# Autodesk Inventor assembly: AdjusterAssembly
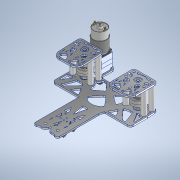
[picture p0: Inventor's stored thumbnail of the model, 180x180]
Saved by Autodesk Inventor 2020.2 (Build 242310000, 310)
## iProperties
Created: 2020-01-19
Part Number: AdjusterAssembly
Document SubType Name: Assembly
Designer: Paul Lefeuvre
Mass: 1604.28 g
Surface Area: 2645.53 cm^2
Volume: 583.424 cm^3
Density: 2.74977 g/cm^3
Author: Paul Lefeuvre
## Documents named in this file (10)
- C:\Users\Paul Lefeuvre\Documents\Inventor\7738-Adjuster\AdjusterAssembly.iam
- C:\Users\Paul Lefeuvre\Documents\Inventor\7738-Adjuster\CaseSheet.ipt
- C:\Users\Paul Lefeuvre\Documents\Inventor\7738-Adjuster\Colson_Performa_1_625_x_0_875_1_2_Hex_bore_217-4045.ipt
- C:\Users\Paul Lefeuvre\Documents\Inventor\7738-Adjuster\Axle1.ipt
- C:\Users\Paul Lefeuvre\Documents\Inventor\7738-Adjuster\F6800_Bearing.ipt
- C:\Users\Paul Lefeuvre\Documents\Inventor\7738-Adjuster\F6801_Bearing.ipt
- C:\Users\Paul Lefeuvre\Documents\Inventor\7738-Adjuster\MainHolder2.ipt
- C:\Users\Paul Lefeuvre\Documents\Inventor\7738-Adjuster\Spacer1.ipt
- C:\Users\Paul Lefeuvre\Documents\Inventor\7738-Adjuster\VersaPlanetary_v1_Single_Stage_10_1_with_775_Series.ipt
- C:\Users\Paul Lefeuvre\Documents\Inventor\7738-Adjuster\Mini V Gantry Kit.ipt
## Components (23 placed, 9 different names)
1. CaseSheet:1 — Insert:11, Mate:2, Mate:3, Mate:4
2. CaseSheet:2 — Insert:12, Insert:48, Insert:49, Insert:50, Insert:51
3. Colson_Performa_1_625_x_0_875_1_2_Hex_bore_217-4045:1 — Angle:1, Insert:2
4. Colson_Performa_1_625_x_0_875_1_2_Hex_bore_217-4045:2 — Angle:2, Insert:6
5. Axle1:1 — Angle:1, Angle:4, Insert:1, Insert:2, Insert:32, Insert:37
6. Axle1:2 — Angle:2, Angle:3, Insert:5, Insert:6, Insert:29, Insert:38
7. F6800_Bearing:1 — Insert:1, Insert:11
8. F6800_Bearing:2 — Insert:5, Insert:12
9. F6801_Bearing:1 — Insert:29
10. F6801_Bearing:2 — Insert:32
11. Colson_Performa_1_625_x_0_875_1_2_Hex_bore_217-4045:3 — Angle:3, Insert:38
12. Colson_Performa_1_625_x_0_875_1_2_Hex_bore_217-4045:4 — Angle:4, Insert:37
13. MainHolder2:1 — Flush:1, Mate:1, Insert:40, Insert:41, Insert:42, Insert:44, Insert:45, Insert:46, Mate:6, Mate:7, Angle:5, Insert:52, Insert:53, Insert:54, Insert:55, Insert:56, Insert:57
14. Spacer1:1 — Insert:40, Mate:3
15. Spacer1:2 — Insert:41, Mate:2
16. Spacer1:3 — Insert:42, Mate:4
17. Spacer1:4 — Insert:49
18. Spacer1:5 — Insert:44, Insert:50
19. Spacer1:6 — Insert:46, Insert:51
20. Spacer1:7 — Insert:52
21. Spacer1:8 — Insert:45, Insert:48
22. VersaPlanetary_v1_Single_Stage_10_1_with_775_Series:1 — Mate:6, Mate:7, Angle:5
23. Mini V Gantry Kit:1 — Insert:53, Insert:54, Insert:55, Insert:56, Insert:57
## Relationships (38: Insert 26, Mate 6, Angle 5, Flush 1)
- Angle:1 (0 deg): Colson_Performa_1_625_x_0_875_1_2_Hex_bore_217-4045:1 ↔ Axle1:1
- Angle:2 (0 deg): Colson_Performa_1_625_x_0_875_1_2_Hex_bore_217-4045:2 ↔ Axle1:2
- Angle:3 (0 deg): Axle1:2 ↔ Colson_Performa_1_625_x_0_875_1_2_Hex_bore_217-4045:3
- Angle:4 (0 deg): Axle1:1 ↔ Colson_Performa_1_625_x_0_875_1_2_Hex_bore_217-4045:4
- Insert:1 (0.6 mm): Axle1:1 ↔ F6800_Bearing:1
- Insert:2 (0.5 mm): Colson_Performa_1_625_x_0_875_1_2_Hex_bore_217-4045:1 ↔ Axle1:1
- Insert:5 (0.6 mm): Axle1:2 ↔ F6800_Bearing:2
- Insert:6 (0.5 mm): Colson_Performa_1_625_x_0_875_1_2_Hex_bore_217-4045:2 ↔ Axle1:2
- Insert:11 (0.6 mm): CaseSheet:1 ↔ F6800_Bearing:1
- Insert:12 (0.6 mm): CaseSheet:2 ↔ F6800_Bearing:2
- Insert:29 (0.6 mm): Axle1:2 ↔ F6801_Bearing:1
- Insert:32 (0.6 mm): Axle1:1 ↔ F6801_Bearing:2
- Insert:37 (0.5 mm): Axle1:1 ↔ Colson_Performa_1_625_x_0_875_1_2_Hex_bore_217-4045:4
- Insert:38 (0.5 mm): Axle1:2 ↔ Colson_Performa_1_625_x_0_875_1_2_Hex_bore_217-4045:3
- Flush:1: MainHolder2:1
- Mate:1: MainHolder2:1
- Insert:40 (0.75 mm): MainHolder2:1 ↔ Spacer1:1
- Insert:41 (0.75 mm): MainHolder2:1 ↔ Spacer1:2
- Insert:42 (0.75 mm): MainHolder2:1 ↔ Spacer1:3
- Insert:44 (0.75 mm): MainHolder2:1 ↔ Spacer1:5
- Mate:2 (0.75 mm): CaseSheet:1 ↔ Spacer1:2
- Mate:3 (0.75 mm): CaseSheet:1 ↔ Spacer1:1
- Mate:4 (0.75 mm): CaseSheet:1 ↔ Spacer1:3
- Insert:45 (0.75 mm): MainHolder2:1 ↔ Spacer1:8
- Insert:46 (0.75 mm): MainHolder2:1 ↔ Spacer1:6
- Insert:48 (0.75 mm): CaseSheet:2 ↔ Spacer1:8
- Insert:49 (0.75 mm): CaseSheet:2 ↔ Spacer1:4
- Insert:50 (0.75 mm): CaseSheet:2 ↔ Spacer1:5
- Insert:51 (0.75 mm): CaseSheet:2 ↔ Spacer1:6
- Mate:6: MainHolder2:1 ↔ VersaPlanetary_v1_Single_Stage_10_1_with_775_Series:1
- Mate:7: MainHolder2:1 ↔ VersaPlanetary_v1_Single_Stage_10_1_with_775_Series:1
- Angle:5 (0 deg): MainHolder2:1 ↔ VersaPlanetary_v1_Single_Stage_10_1_with_775_Series:1
- Insert:52 (0.75 mm): MainHolder2:1 ↔ Spacer1:7
- Insert:53 (0.6 mm): MainHolder2:1 ↔ Mini V Gantry Kit:1
- Insert:54 (0.6 mm): MainHolder2:1 ↔ Mini V Gantry Kit:1
- Insert:55 (0.6 mm): MainHolder2:1 ↔ Mini V Gantry Kit:1
- Insert:56 (0.6 mm): MainHolder2:1 ↔ Mini V Gantry Kit:1
- Insert:57 (0.6 mm): MainHolder2:1 ↔ Mini V Gantry Kit:1
